# Autodesk Inventor assembly: Shelf Holder Joint
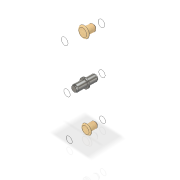
[picture p0: Inventor's stored thumbnail of the model, 180x180]
Saved by Autodesk Inventor 2024.3 (Build 283343000, 343)
## iProperties
RuleStatus: InUse
Created: 2023-02-06
Part Number: Shelf Holder Joint
Document SubType Name: Assembly
Designer: sauliusd
Author: sauliusd
## Documents named in this file (4)
- C:\W4INV 2024 Design\SMART HARDWARE\Shelf Holder\Shelf Holder Joint.iam
- C:\W4INV 2024 Design\SMART HARDWARE\Shelf Holder\Parts\Shelf Holder.ipt
- C:\W4INV 2024 Design\_LIBRARY\Shelf holder D5\Shelf support D5 L16 with hole covers.ipt
- C:\W4INV 2024 Design\LIBRARY\Holders\Shelf holder D5.ipt
## Components (3 placed, 3 different names)
1. @Skeleton — Flush:1, Flush:2, Flush:3, Insert:1
2. Shelf Support D5 — Insert:1, Angle:1
3. Shelf support D5 L16 with hole covers:2
## Component patterns: (2 elements, first: Shelf Support D5)
## Relationships (5: Flush 3, Insert 1, Angle 1)
- Flush:1: @Skeleton
- Flush:2: @Skeleton
- Flush:3: @Skeleton
- Insert:1: @Skeleton ↔ Shelf Support D5
- Angle:1 (0 deg): Shelf Support D5
## Named parameters: ContactPatchHeight = 18 mm, ContactPatchWidth = 500 mm, PillarBoardT = 18 mm, HoleNumber = 3, ShiftFromSide1 = 60 mm, ShiftFromSide2 = 60 mm, MaxAllowedDistance = 500 mm, MinAllowedDistance = 20 mm
